# Autodesk Inventor assembly: endcapLeft
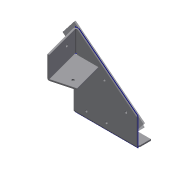
[picture p0: Inventor's stored thumbnail of the model, 180x180]
Saved by Autodesk Inventor 2016 (Build 200138000, 138)
## iProperties
Created: 2015-05-12
Part Number: endcapLeft
Document SubType Name: Assembly
Designer: krosie
Author: krosie
## Documents named in this file (5)
- C:\Users\krosie\Google Drive\HERA\hera-cad\support\endcaps\lasercutOption.iam
- endCapOptionLeft.iam
- C:\Users\krosie\Google Drive\HERA\hera-cad\support\endcapOptionLeft.ipt
- C:\Users\krosie\Google Drive\HERA\hera-cad\support\endcapOptionLeftAngle.ipt
- C:\Users\krosie\Google Drive\HERA\hera-cad\support\endcaps\EndcapSpacer.ipt
## Components (3 placed, 3 different names)
1. endcapOptionLeft:1 — Flush:1, Mate:1, Mate:2, Mate:3, Mate:4, Insert:1
2. endcapOptionLeftAngle:1 — Flush:1, Mate:1, Mate:2
3. EndcapSpacer:1 — Mate:3, Mate:4, Insert:1
## Relationships (6: Mate 4, Flush 1, Insert 1)
- Flush:1: endcapOptionLeft:1 ↔ endcapOptionLeftAngle:1
- Mate:1: endcapOptionLeft:1 ↔ endcapOptionLeftAngle:1
- Mate:2: endcapOptionLeft:1 ↔ endcapOptionLeftAngle:1
- Mate:3: endcapOptionLeft:1 ↔ EndcapSpacer:1
- Mate:4: endcapOptionLeft:1 ↔ EndcapSpacer:1
- Insert:1: endcapOptionLeft:1 ↔ EndcapSpacer:1
